# Autodesk Inventor assembly: triangle_brace
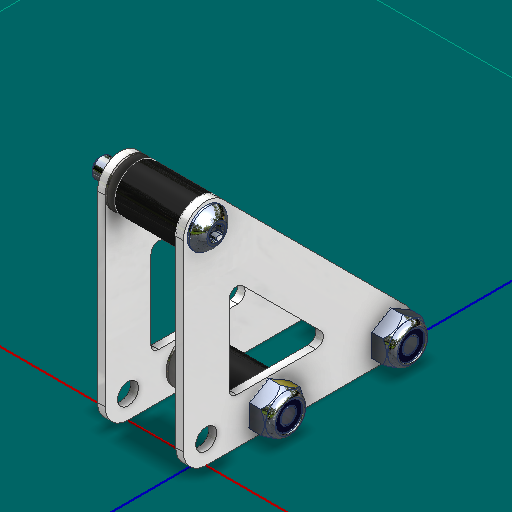
[picture p0: Inventor's stored thumbnail of the model, 512x512]
Saved by Autodesk Inventor 2025 (Build 290162000, 162)
## iProperties
Created: 2024-08-19
Part Number: triangle_brace
Document SubType Name: Assembly
Designer: averey
Author: averey
## Documents named in this file (9)
- C:\Users\avere\vex_robotics_high_stakes\hardware\cad\ATLAS\tower\structure\triangle_brace.iam
- C:\Users\avere\vex_robotics_high_stakes\hardware\cad\ATLAS\chassis\structure\custom_parts\right_angle_gusset.ipt
- C:\Users\avere\vex_robotics_high_stakes\hardware\cad\VEX-CAD-Inventor\Motion\Spacers\Spacer Nylon .375 OD.ipt
- C:\Users\avere\vex_robotics_high_stakes\hardware\cad\VEX-CAD-Inventor\Motion\Spacers\Spacer Nylon .375 OD\NSpacer .375 OD x .500.ipt
- C:\Users\avere\vex_robotics_high_stakes\hardware\cad\VEX-CAD-Inventor\Motion\Spacers\Washer Steel\SWasher .375 OD x .015625.ipt
- C:\Users\avere\vex_robotics_high_stakes\hardware\cad\VEX-CAD-Inventor\Motion\Spacers\Washer Steel.ipt
- C:\Users\avere\vex_robotics_high_stakes\hardware\cad\VEX-CAD-Inventor\Structure\Hardware\Screw Steel - Star\SScrew Star Smooth .875.ipt
- C:\Users\avere\vex_robotics_high_stakes\hardware\cad\VEX-CAD-Inventor\Structure\Hardware\Screw Steel - Star.ipt
- C:\Users\avere\vex_robotics_high_stakes\hardware\cad\VEX-CAD-Inventor\Structure\Hardware\Nut Thin Nylock.ipt
## Components (13 placed, 5 different names)
1. right_angle_gusset:1 — Insert:1, Insert:5, Insert:6, Insert:7, Insert:9, Insert:10
2. right_angle_gusset:2 — Insert:1, Mate:2, Insert:2, Insert:3, Insert:4, Insert:11, Insert:12, Insert:13
3. NSpacer .375 OD x .500:2 — Insert:2
4. NSpacer .375 OD x .500:3 — Insert:3
5. NSpacer .375 OD x .500:4 — Insert:4
6. SWasher .375 OD x .015625:1 — Insert:5
7. SWasher .375 OD x .015625:2 — Insert:6
8. SWasher .375 OD x .015625:3 — Insert:7
9. SScrew Star Smooth .875:1 — Insert:13
10. SScrew Star Smooth .875:2 — Insert:9
11. SScrew Star Smooth .875:3 — Insert:10
12. Nut Thin Nylock:1 — Insert:11
13. Nut Thin Nylock:2 — Insert:12
## Relationships (14: Insert 12, Mate 2)
- [Mate]: right_angle_gusset:1 ↔ right_angle_gusset:2
- Insert:1 (14.6844 mm): right_angle_gusset:1 ↔ right_angle_gusset:2
- Mate:2: right_angle_gusset:2
- Insert:2: right_angle_gusset:2 ↔ NSpacer .375 OD x .500:2
- Insert:3: right_angle_gusset:2 ↔ NSpacer .375 OD x .500:3
- Insert:4: right_angle_gusset:2 ↔ NSpacer .375 OD x .500:4
- Insert:5: right_angle_gusset:1 ↔ SWasher .375 OD x .015625:1
- Insert:6: right_angle_gusset:1 ↔ SWasher .375 OD x .015625:2
- Insert:7: right_angle_gusset:1 ↔ SWasher .375 OD x .015625:3
- Insert:9: right_angle_gusset:1 ↔ SScrew Star Smooth .875:2
- Insert:10: right_angle_gusset:1 ↔ SScrew Star Smooth .875:3
- Insert:11: right_angle_gusset:2 ↔ Nut Thin Nylock:1
- Insert:12: right_angle_gusset:2 ↔ Nut Thin Nylock:2
- Insert:13: right_angle_gusset:2 ↔ SScrew Star Smooth .875:1
## Named parameters: d65_d212 = 0 mm
